# Autodesk Inventor assembly: Outer Shield
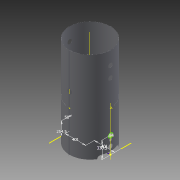
[picture p0: Inventor's stored thumbnail of the model, 180x180]
Saved by Autodesk Inventor 2015 (Build 190159000, 159)
## iProperties
Created: 2014-06-19
Part Number: Outer Shield
Document SubType Name: Assembly
Designer: Aki
Author: Aki
## Documents named in this file (5)
- C:\ColdMatter\CADFiles\EDM Machine\EDM Outer Shield\Outer Shield.iam
- C:\ColdMatter\CADFiles\EDM Machine\EDM Outer Shield\Lower Front Half.ipt
- C:\ColdMatter\CADFiles\EDM Machine\EDM Outer Shield\Lower Back Half.ipt
- C:\ColdMatter\CADFiles\EDM Machine\EDM Outer Shield\Upper Front Half New.ipt
- C:\ColdMatter\CADFiles\EDM Machine\EDM Outer Shield\Upper Back Half New.ipt
## Components (4 placed, 4 different names)
1. Lower Front Half:1 — Mate:1, Mate:2, Mate:3, Mate:4, Mate:21, Mate:24, Mate:25
2. Lower Back Half:1 — Mate:2, Mate:3, Mate:4, Mate:25
3. Upper Front Half New:2 — Mate:21, Mate:26, Mate:27, Mate:28
4. Upper Back Half New:1 — Mate:26, Mate:27, Mate:28
## Relationships (10: Mate 10)
- Mate:1: Lower Front Half:1
- Mate:2: Lower Front Half:1 ↔ Lower Back Half:1
- Mate:3: Lower Front Half:1 ↔ Lower Back Half:1
- Mate:4: Lower Front Half:1 ↔ Lower Back Half:1
- Mate:21: Lower Front Half:1 ↔ Upper Front Half New:2
- Mate:24: Lower Front Half:1
- Mate:25: Lower Front Half:1 ↔ Lower Back Half:1
- Mate:26: Upper Front Half New:2 ↔ Upper Back Half New:1
- Mate:27: Upper Front Half New:2 ↔ Upper Back Half New:1
- Mate:28: Upper Front Half New:2 ↔ Upper Back Half New:1
